# Autodesk Inventor assembly: BG302_trajan20_21
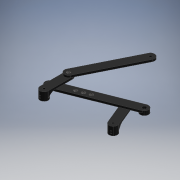
[picture p0: Inventor's stored thumbnail of the model, 180x180]
Saved by Autodesk Inventor 2022.2 (Build 262287000, 287)
## iProperties
Company: HTBLA Kaindorf
RuleStatus: InUse
Created: 2022-09-14
Part Number: BG302_trajan20_21
Project: Zeichenmaschine_v2_a
Material: Generisch
Description: gelenke_neu
Document SubType Name: Assembly
Designer: trajan20
AfterDocNew0: iProperties-Editor_aufrufen
Author: jan
Keywords: 2021
## Documents named in this file (5)
- C:\Users\jan\Documents\DrawMachine\DrawMachineConstruction\Projekt\Zeichenmaschine_v2\BG302_trajan20_21_Zeichenmaschine_v2_a_gelenke_neu.iam
- C:\Users\jan\Documents\DrawMachine\DrawMachineConstruction\Projekt\Zeichenmaschine_v2\BT301_trajan20_21_Zeichenmaschine_v2_gelenk 1.ipt
- C:\Users\jan\Documents\DrawMachine\DrawMachineConstruction\Projekt\Zeichenmaschine_v2\BT301_trajan20_21_Zeichenmaschine_v2_gelenk a.ipt
- C:\Users\jan\Documents\DrawMachine\DrawMachineConstruction\Projekt\Zeichenmaschine_v2\DIN 625 SKF - SKF 628_5-2Z_5x10x4.ipt
- C:\Users\jan\Documents\DrawMachine\DrawMachineConstruction\Projekt\Zeichenmaschine_v2\BT303_trajan20_21_Zeichenmaschine_v2_gelenk b.ipt
## Components (9 placed, 4 different names)
1. BT301_trajan20_21_Zeichenmaschine_v2_gelenk 1:1 — Passend:1, Passend:4, Passend:5
2. BT301_trajan20_21_Zeichenmaschine_v2_gelenk 1:2 — Passend:5, Passend:6
3. BT301_trajan20_21_Zeichenmaschine_v2_gelenk a:1 — Passend:1, Passend:2, Passend:3
4. DIN 625 SKF- beidseitig abgedeckt SKF 628/5-2Z:1 — Passend:2, Passend:3, Passend:4
5. BT303_trajan20_21_Zeichenmaschine_v2_gelenk b:1 — Passend:6, Passend:7, Passend:8, Passend:9, Passend:10, Passend:11, Passend:12, Passend:13, Passend:14
6. DIN 625 SKF- beidseitig abgedeckt SKF 628/5-2Z:2 — Passend:7, Passend:8
7. DIN 625 SKF- beidseitig abgedeckt SKF 628/5-2Z:3 — Passend:13, Passend:14
8. DIN 625 SKF- beidseitig abgedeckt SKF 628/5-2Z:4 — Passend:11, Passend:12
9. DIN 625 SKF- beidseitig abgedeckt SKF 628/5-2Z:5 — Passend:9, Passend:10
## Relationships (14: Mate 14)
- Passend:1 [Mate]: BT301_trajan20_21_Zeichenmaschine_v2_gelenk 1:1 ↔ BT301_trajan20_21_Zeichenmaschine_v2_gelenk a:1
- Passend:2 [Mate]: BT301_trajan20_21_Zeichenmaschine_v2_gelenk a:1 ↔ DIN 625 SKF- beidseitig abgedeckt SKF 628/5-2Z:1
- Passend:3 [Mate]: BT301_trajan20_21_Zeichenmaschine_v2_gelenk a:1 ↔ DIN 625 SKF- beidseitig abgedeckt SKF 628/5-2Z:1
- Passend:4 [Mate]: BT301_trajan20_21_Zeichenmaschine_v2_gelenk 1:1 ↔ DIN 625 SKF- beidseitig abgedeckt SKF 628/5-2Z:1
- Passend:5 [Mate] (120 mm): BT301_trajan20_21_Zeichenmaschine_v2_gelenk 1:1 ↔ BT301_trajan20_21_Zeichenmaschine_v2_gelenk 1:2
- Passend:6 [Mate]: BT301_trajan20_21_Zeichenmaschine_v2_gelenk 1:2 ↔ BT303_trajan20_21_Zeichenmaschine_v2_gelenk b:1
- Passend:7 [Mate]: BT303_trajan20_21_Zeichenmaschine_v2_gelenk b:1 ↔ DIN 625 SKF- beidseitig abgedeckt SKF 628/5-2Z:2
- Passend:8 [Mate]: BT303_trajan20_21_Zeichenmaschine_v2_gelenk b:1 ↔ DIN 625 SKF- beidseitig abgedeckt SKF 628/5-2Z:2
- Passend:9 [Mate]: BT303_trajan20_21_Zeichenmaschine_v2_gelenk b:1 ↔ DIN 625 SKF- beidseitig abgedeckt SKF 628/5-2Z:5
- Passend:10 [Mate]: BT303_trajan20_21_Zeichenmaschine_v2_gelenk b:1 ↔ DIN 625 SKF- beidseitig abgedeckt SKF 628/5-2Z:5
- Passend:11 [Mate]: BT303_trajan20_21_Zeichenmaschine_v2_gelenk b:1 ↔ DIN 625 SKF- beidseitig abgedeckt SKF 628/5-2Z:4
- Passend:12 [Mate]: BT303_trajan20_21_Zeichenmaschine_v2_gelenk b:1 ↔ DIN 625 SKF- beidseitig abgedeckt SKF 628/5-2Z:4
- Passend:13 [Mate]: BT303_trajan20_21_Zeichenmaschine_v2_gelenk b:1 ↔ DIN 625 SKF- beidseitig abgedeckt SKF 628/5-2Z:3
- Passend:14 [Mate]: BT303_trajan20_21_Zeichenmaschine_v2_gelenk b:1 ↔ DIN 625 SKF- beidseitig abgedeckt SKF 628/5-2Z:3
